# Autodesk Inventor assembly: Frame 1647030135921
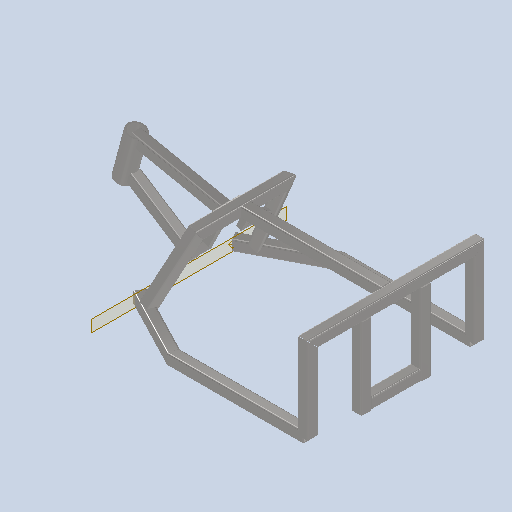
[picture p0: Inventor's stored thumbnail of the model, 512x512]
Saved by Autodesk Inventor 2022.2 (Build 262287000, 287)
## iProperties
_FrameDoc: Frame Assembly
_Version: 25.0.0
Created: 2022-03-11
Part Number: Frame 1647030135921
Document SubType Name: Assembly
Designer: foriw
Mass: 2723.63 g
Surface Area: 3396.09 cm^2
Volume: 346.96 cm^3
Density: 7.85 g/cm^3
Author: foriw
## Documents named in this file (21)
- C:\Users\foriw\OneDrive\Dokumenter\Inventor\Beercart - Meaktroronik - new\beercart assembly - mekatronik\Frame\Frame 1647030135921.iam
- C:\Users\foriw\OneDrive\Dokumenter\Inventor\Beercart - Meaktroronik - new\beercart assembly - mekatronik\Frame\Skeleton 1647030135922.ipt
- C:\Users\foriw\OneDrive\Dokumenter\Inventor\Beercart - Meaktroronik - new\beercart assembly - mekatronik\Frame\ISO 12633-2 20x20x2 1647030137505.ipt
- C:\Users\foriw\OneDrive\Dokumenter\Inventor\Beercart - Meaktroronik - new\beercart assembly - mekatronik\Frame\ISO 12633-2 20x20x2 1647030137863.ipt
- C:\Users\foriw\OneDrive\Dokumenter\Inventor\Beercart - Meaktroronik - new\beercart assembly - mekatronik\Frame\ISO 12633-2 20x20x2 1647030137981.ipt
- C:\Users\foriw\OneDrive\Dokumenter\Inventor\Beercart - Meaktroronik - new\beercart assembly - mekatronik\Frame\ISO 12633-2 20x20x2 1647030138110.ipt
- C:\Users\foriw\OneDrive\Dokumenter\Inventor\Beercart - Meaktroronik - new\beercart assembly - mekatronik\Frame\ISO 12633-2 20x20x2 1647030138225.ipt
- C:\Users\foriw\OneDrive\Dokumenter\Inventor\Beercart - Meaktroronik - new\beercart assembly - mekatronik\Frame\ISO 12633-2 20x20x2 1647030639616.ipt
- C:\Users\foriw\OneDrive\Dokumenter\Inventor\Beercart - Meaktroronik - new\beercart assembly - mekatronik\Frame\ISO 12633-2 20x20x2 1647030639707.ipt
- C:\Users\foriw\OneDrive\Dokumenter\Inventor\Beercart - Meaktroronik - new\beercart assembly - mekatronik\Frame\ISO 1035_2 10x 10 1647602095470.ipt
- C:\Users\foriw\OneDrive\Dokumenter\Inventor\Beercart - Meaktroronik - new\beercart assembly - mekatronik\Frame\ISO 1035_2 10x 10 1647602096505.ipt
- C:\Users\foriw\OneDrive\Dokumenter\Inventor\Beercart - Meaktroronik - new\beercart assembly - mekatronik\Frame\ISO 1035_2 10x 10 1647602096566.ipt
- C:\Users\foriw\OneDrive\Dokumenter\Inventor\Beercart - Meaktroronik - new\beercart assembly - mekatronik\Frame\ISO 1035_2 10x 10 1647602096620.ipt
- C:\Users\foriw\OneDrive\Dokumenter\Inventor\Beercart - Meaktroronik - new\beercart assembly - mekatronik\Frame\ISO 12633-2 20x20x2 1647606064149.ipt
- C:\Users\foriw\OneDrive\Dokumenter\Inventor\Beercart - Meaktroronik - new\beercart assembly - mekatronik\Frame\ISO 12633-2 20x20x2 1647606064205.ipt
- C:\Users\foriw\OneDrive\Dokumenter\Inventor\Beercart - Meaktroronik - new\beercart assembly - mekatronik\Frame\ISO 12633-2 20x20x2 1647606177319.ipt
- C:\Users\foriw\OneDrive\Dokumenter\Inventor\Beercart - Meaktroronik - new\beercart assembly - mekatronik\Frame\ISO 12633-2 20x20x2 1647606177438.ipt
- C:\Users\foriw\OneDrive\Dokumenter\Inventor\Beercart - Meaktroronik - new\beercart assembly - mekatronik\Frame\ISO 12633-2 20x20x2 1648114433069.ipt
- C:\Users\foriw\OneDrive\Dokumenter\Inventor\Beercart - Meaktroronik - new\beercart assembly - mekatronik\Frame\ISO 12633-2 20x20x2 1648114433206.ipt
- C:\Users\foriw\OneDrive\Dokumenter\Inventor\Beercart - Meaktroronik - new\beercart assembly - mekatronik\Frame\FrontWheelFrame.iam
- C:\Users\foriw\OneDrive\Dokumenter\Inventor\Beercart - Meaktroronik - new\beercart assembly - mekatronik\Frame\ISO 12633-2 20x20x2 1648165831228.ipt
## Components (20 placed, 15 different names)
1. Reference Skeleton
2. ISO 12633-2 20x20x2 - 329.48:2
3. ISO 12633-2 20x20x2 - 159,65:1
4. ISO 12633-2 20x20x2 - 159,65:2
5. ISO 12633-2 20x20x2 - 260:1
6. ISO 12633-2 20x20x2 - 185.3:3
7. ISO 12633-2 20x20x2 - 178.64:1
8. ISO 12633-2 20x20x2 - 178.64:2
9. ISO 1035/2 10x 10 - 63.19:1
10. ISO 1035/2 10x 10 - 63.31:1
11. ISO 1035/2 10x 10 - 44.25:1
12. ISO 1035/2 10x 10 - 44.22:2
13. ISO 12633-2 20x20x2 - 252.18:1
14. ISO 12633-2 20x20x2 - 252.18:2
15. ISO 12633-2 20x20x2 - 148.66:1 — Mate:1, Mate:3
16. ISO 12633-2 20x20x2 - 148.66:2 — Mate:2, Mate:4, Mate:5
17. ISO 12633-2 20x20x2 - 150:1
18. ISO 12633-2 20x20x2 - 150:2
19. FrontWheelFrame:1 [sub-assembly]
20. ISO 12633-2 20x20x2 - 90:1
## Relationships (5: Mate 5)
- Mate:1: ISO 12633-2 20x20x2 - 148.66:1
- Mate:2: ISO 12633-2 20x20x2 - 148.66:2
- Mate:3: ISO 12633-2 20x20x2 - 148.66:1
- Mate:4: ISO 12633-2 20x20x2 - 148.66:2
- Mate:5: ISO 12633-2 20x20x2 - 148.66:2
